# Autodesk Inventor assembly: Leg_joint_roll_pitch
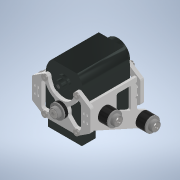
[picture p0: Inventor's stored thumbnail of the model, 180x180]
Saved by Autodesk Inventor 2020 (Build 240168000, 168)
## iProperties
Part Number: Leg_joint_roll_pitch
Document SubType Name: Assembly
Designer: Masato Kubotera
Mass: 155.537 g
Surface Area: 333.044 cm^2
Volume: 75.5065 cm^3
Density: 2.05992 g/cm^3
Author: Masato Kubotera
## Documents named in this file (20)
- C:\Users\Masato\Documents\Inventor\CIT Brains_Inventor\OpenPlatform_ver3_0\LowerBody\Leg_joit\Leg_joint_roll_pitch.iam
- C:\Users\Masato\Documents\Inventor\CIT Brains_Inventor\OpenPlatform_ver3_0\LowerBody\Leg_joit\Leg_joint_pitch_frame.ipt
- C:\Users\Masato\Documents\Inventor\CIT Brains_Inventor\OpenPlatform_ver3_0\LowerBody\Leg_joit\Leg_joint_roll_front_frame.ipt
- C:\Users\Masato\Documents\Inventor\CIT Brains_Inventor\OpenPlatform_ver3_0\Ready_Made\B3M11xx.ipt
- C:\Users\Masato\Documents\Inventor\CIT Brains_Inventor\OpenPlatform_ver3_0\Ready_Made\SLSBF6-39_5-M3-N3.ipt
- C:\Users\Masato\Documents\Inventor\CIT Brains_Inventor\OpenPlatform_ver3_0\Ready_Made\UUW-0312-10BH.ipt
- C:\Users\Masato\Documents\Inventor\CIT Brains_Inventor\OpenPlatform_ver3_0\Ready_Made\BRU-311S.ipt
- C:\Users\Masato\Documents\Inventor\CIT Brains_Inventor\OpenPlatform_ver3_0\Ready_Made\Screw\M3-6.ipt
- C:\Users\Masato\Documents\Inventor\CIT Brains_Inventor\OpenPlatform_ver3_0\Ready_Made\Screw\M2_6-20.ipt
- C:\Users\Masato\Documents\Inventor\CIT Brains_Inventor\OpenPlatform_ver3_0\Ready_Made\Screw\M2_6-15.ipt
- C:\Users\Masato\Documents\Inventor\CIT Brains_Inventor\OpenPlatform_ver3_0\Ready_Made\80F-0603.ipt
- C:\Users\Masato\Documents\Inventor\CIT Brains_Inventor\OpenPlatform_ver3_0\Ready_Made\CC-0612-15B.ipt
- C:\Users\Masato\Documents\Inventor\CIT Brains_Inventor\OpenPlatform_ver3_0\Ready_Made\CC-0612-50B.ipt
- C:\Users\Masato\Documents\Inventor\CIT Brains_Inventor\OpenPlatform_ver3_0\Ready_Made\SF319.ipt
- C:\Users\Masato\Documents\Inventor\CIT Brains_Inventor\OpenPlatform_ver3_0\Ready_Made\S3-07-3W.ipt
- C:\Users\Masato\Documents\Inventor\CIT Brains_Inventor\OpenPlatform_ver3_0\LowerBody\Leg_joit\Leg_joint_roll_back_frame.ipt
- C:\Users\Masato\Documents\Inventor\CIT Brains_Inventor\OpenPlatform_ver3_0\Ready_Made\ARU-306S.ipt
- ARU-306S.ipt
- C:\Users\Masato\Documents\Inventor\CIT Brains_Inventor\OpenPlatform_ver3_0\Ready_Made\ARU-309_5S.ipt
- ARU-309_5S.ipt
## Components (46 placed, 17 different names)
1. Leg_joint_pitch_frame:1 — フラッシュ:1, 挿入:11, 挿入:27, 挿入:28, 挿入:133
2. Leg_joint_pitch_frame:2 — 挿入:12, 挿入:25, 挿入:26, フラッシュ:1, 挿入:132, メイト:11, メイト:12, フラッシュ:7
3. B3M11xx:1 — フラッシュ:6, メイト:8, メイト:10, 挿入:152, 挿入:153, 挿入:154, 挿入:155, 挿入:162, 挿入:163, 挿入:164, 挿入:165
4. SLSBF6-39_5-M3-N3:1 — 挿入:11, 挿入:12
5. UUW-0312-10BH:1 — 挿入:27, 挿入:100, 挿入:124
6. UUW-0312-10BH:2 — 挿入:28, 挿入:101, 挿入:125
7. UUW-0312-10BH:3 — 挿入:25, 挿入:99, 挿入:126
8. UUW-0312-10BH:4 — 挿入:26, 挿入:98, 挿入:127
9. UUW-0312-10BH:5 — 挿入:170, 挿入:172, 挿入:174
10. UUW-0312-10BH:6 — 挿入:120, 挿入:156, 挿入:171
11. BRU-311S:1 — 挿入:99
12. BRU-311S:2 — 挿入:98
13. BRU-311S:3 — 挿入:101
14. BRU-311S:4 — 挿入:100
15. M3-6:2 — 挿入:161
16. M2_6-20:1 — 挿入:157
17. M2_6-20:2 — 挿入:159
18. M2_6-20:3 — 挿入:158
19. M2_6-20:4 — 挿入:160
20. M2_6-15:1 — 挿入:168
21. M2_6-15:2 — 挿入:169
22. M2_6-15:3 — 挿入:167
23. M2_6-15:4 — 挿入:166
24. 80F-0603:1 — 挿入:134
25. 80F-0603:3 — 挿入:130
26. 80F-0603:4 — 挿入:131
27. 80F-0603:5 — 挿入:129
28. 80F-0603:6 — 挿入:128
29. CC-0612-15B:1 — 挿入:114, 挿入:124
30. CC-0612-15B:2 — 挿入:115, 挿入:125
31. CC-0612-15B:3 — 挿入:116, 挿入:127
32. CC-0612-15B:4 — 挿入:117, 挿入:126
33. CC-0612-15B:5 — 挿入:120, 挿入:134
34. CC-0612-50B:1 — 挿入:114, 挿入:130
35. CC-0612-50B:2 — 挿入:115, 挿入:131
36. CC-0612-50B:3 — 挿入:116, 挿入:128
37. CC-0612-50B:4 — 挿入:117, 挿入:129
38. SF319:1 — 挿入:132
39. SF319:2 — 挿入:133
40. S3-07-3W:1 — 角度:1, 挿入:151
41. Leg_joint_roll_back_frame:1 — 挿入:161, 挿入:162, 挿入:163, 挿入:164, 挿入:165, 挿入:166, 挿入:167, 挿入:168, 挿入:169, 挿入:170
42. Leg_joint_roll_front_frame:1 — 角度:1, 挿入:151, 挿入:152, 挿入:153, 挿入:154, 挿入:155, 挿入:156, 挿入:157, 挿入:158, 挿入:159, 挿入:160, メイト:11, メイト:12, フラッシュ:7
43. ARU-306S:1 — 挿入:171
44. CC-0612-50B:5 — 挿入:172, 挿入:173
45. 80F-0603:7 — 挿入:173
46. ARU-309_5S:1 — 挿入:174
## Relationships (58: Insert 50, Mate 4, Flush 3, Angle 1)
- フラッシュ:1 [Flush]: Leg_joint_pitch_frame:1 ↔ Leg_joint_pitch_frame:2
- 挿入:11 [Insert]: Leg_joint_pitch_frame:1 ↔ SLSBF6-39_5-M3-N3:1
- 挿入:12 [Insert]: Leg_joint_pitch_frame:2 ↔ SLSBF6-39_5-M3-N3:1
- 挿入:25 [Insert]: Leg_joint_pitch_frame:2 ↔ UUW-0312-10BH:3
- 挿入:26 [Insert]: Leg_joint_pitch_frame:2 ↔ UUW-0312-10BH:4
- 挿入:27 [Insert]: Leg_joint_pitch_frame:1 ↔ UUW-0312-10BH:1
- 挿入:28 [Insert]: Leg_joint_pitch_frame:1 ↔ UUW-0312-10BH:2
- フラッシュ:6 [Flush]: B3M11xx:1
- メイト:8 [Mate]: B3M11xx:1
- メイト:10 [Mate]: B3M11xx:1
- 挿入:98 [Insert]: UUW-0312-10BH:4 ↔ BRU-311S:2
- 挿入:99 [Insert]: UUW-0312-10BH:3 ↔ BRU-311S:1
- 挿入:100 [Insert]: UUW-0312-10BH:1 ↔ BRU-311S:4
- 挿入:101 [Insert]: UUW-0312-10BH:2 ↔ BRU-311S:3
- 挿入:114 [Insert]: CC-0612-15B:1 ↔ CC-0612-50B:1
- 挿入:115 [Insert]: CC-0612-15B:2 ↔ CC-0612-50B:2
- 挿入:116 [Insert]: CC-0612-15B:3 ↔ CC-0612-50B:3
- 挿入:117 [Insert]: CC-0612-15B:4 ↔ CC-0612-50B:4
- 挿入:120 [Insert]: UUW-0312-10BH:6 ↔ CC-0612-15B:5
- 挿入:124 [Insert]: UUW-0312-10BH:1 ↔ CC-0612-15B:1
- 挿入:125 [Insert]: UUW-0312-10BH:2 ↔ CC-0612-15B:2
- 挿入:126 [Insert]: UUW-0312-10BH:3 ↔ CC-0612-15B:4
- 挿入:127 [Insert]: UUW-0312-10BH:4 ↔ CC-0612-15B:3
- 挿入:128 [Insert]: 80F-0603:6 ↔ CC-0612-50B:3
- 挿入:129 [Insert]: 80F-0603:5 ↔ CC-0612-50B:4
- 挿入:130 [Insert]: 80F-0603:3 ↔ CC-0612-50B:1
- 挿入:131 [Insert]: 80F-0603:4 ↔ CC-0612-50B:2
- 挿入:132 [Insert]: Leg_joint_pitch_frame:2 ↔ SF319:1
- 挿入:133 [Insert]: Leg_joint_pitch_frame:1 ↔ SF319:2
- 挿入:134 [Insert]: 80F-0603:1 ↔ CC-0612-15B:5
- 角度:1 [Angle] (0 deg): S3-07-3W:1 ↔ Leg_joint_roll_front_frame:1
- 挿入:151 [Insert]: S3-07-3W:1 ↔ Leg_joint_roll_front_frame:1
- 挿入:152 [Insert]: B3M11xx:1 ↔ Leg_joint_roll_front_frame:1
- 挿入:153 [Insert]: B3M11xx:1 ↔ Leg_joint_roll_front_frame:1
- 挿入:154 [Insert]: B3M11xx:1 ↔ Leg_joint_roll_front_frame:1
- 挿入:155 [Insert]: B3M11xx:1 ↔ Leg_joint_roll_front_frame:1
- 挿入:156 [Insert]: UUW-0312-10BH:6 ↔ Leg_joint_roll_front_frame:1
- 挿入:157 [Insert]: M2_6-20:1 ↔ Leg_joint_roll_front_frame:1
- 挿入:158 [Insert]: M2_6-20:3 ↔ Leg_joint_roll_front_frame:1
- 挿入:159 [Insert]: M2_6-20:2 ↔ Leg_joint_roll_front_frame:1
- 挿入:160 [Insert]: M2_6-20:4 ↔ Leg_joint_roll_front_frame:1
- メイト:11 [Mate] (0.01 mm): Leg_joint_pitch_frame:2 ↔ Leg_joint_roll_front_frame:1
- メイト:12 [Mate] (0.01 mm): Leg_joint_pitch_frame:2 ↔ Leg_joint_roll_front_frame:1
- フラッシュ:7 [Flush]: Leg_joint_pitch_frame:2 ↔ Leg_joint_roll_front_frame:1
- 挿入:161 [Insert]: M3-6:2 ↔ Leg_joint_roll_back_frame:1
- 挿入:162 [Insert]: B3M11xx:1 ↔ Leg_joint_roll_back_frame:1
- 挿入:163 [Insert]: B3M11xx:1 ↔ Leg_joint_roll_back_frame:1
- 挿入:164 [Insert]: B3M11xx:1 ↔ Leg_joint_roll_back_frame:1
- 挿入:165 [Insert]: B3M11xx:1 ↔ Leg_joint_roll_back_frame:1
- 挿入:166 [Insert]: M2_6-15:4 ↔ Leg_joint_roll_back_frame:1
- 挿入:167 [Insert]: M2_6-15:3 ↔ Leg_joint_roll_back_frame:1
- 挿入:168 [Insert]: M2_6-15:1 ↔ Leg_joint_roll_back_frame:1
- 挿入:169 [Insert]: M2_6-15:2 ↔ Leg_joint_roll_back_frame:1
- 挿入:170 [Insert]: UUW-0312-10BH:5 ↔ Leg_joint_roll_back_frame:1
- 挿入:171 [Insert]: UUW-0312-10BH:6 ↔ ARU-306S:1
- 挿入:172 [Insert]: UUW-0312-10BH:5 ↔ CC-0612-50B:5
- 挿入:173 [Insert]: CC-0612-50B:5 ↔ 80F-0603:7
- 挿入:174 [Insert]: UUW-0312-10BH:5 ↔ ARU-309_5S:1
